# Autodesk Inventor assembly: DribblerUnit
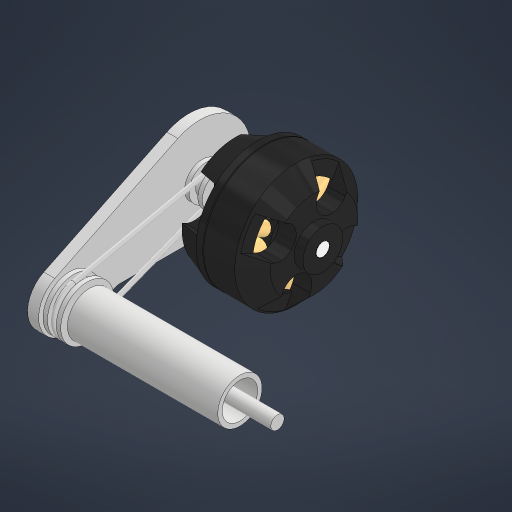
[picture p0: Inventor's stored thumbnail of the model, 512x512]
Saved by Autodesk Inventor 2024.2 (Build 282272000, 272)
## iProperties
Created: 2023-12-27
Part Number: DribblerUnit
Document SubType Name: Assembly
Designer: Hanaoka
Author: Hanaoka
## Documents named in this file (9)
- G:\共有ドライブ\reRo\05_個人\hanaoka\inventor\DribblerUnit\DribblerUnit.iam
- G:\共有ドライブ\reRo\05_個人\hanaoka\inventor\DribblerUnit\Gear_Cover.ipt
- G:\共有ドライブ\reRo\05_個人\hanaoka\inventor\DribblerUnit\Bearing_C-FL673ZZ.ipt
- G:\共有ドライブ\reRo\05_個人\hanaoka\inventor\DribblerUnit\Shaft.ipt
- G:\共有ドライブ\reRo\05_個人\hanaoka\inventor\DribblerUnit\tube.ipt
- G:\共有ドライブ\reRo\05_個人\hanaoka\inventor\DribblerUnit\C2822 1400KV BLDC v25\C2822 1400KV BLDC v25.ipt
- G:\共有ドライブ\reRo\05_個人\hanaoka\inventor\DribblerUnit\Pulley_S.ipt
- G:\共有ドライブ\reRo\05_個人\hanaoka\inventor\DribblerUnit\Pulley_L.ipt
- G:\共有ドライブ\reRo\05_個人\hanaoka\inventor\DribblerUnit\Belt.ipt
## Components (8 placed, 8 different names)
1. Gear_Cover:1 — 挿入:1, 挿入:2, 挿入:4, 挿入:5
2. Bearing_C-FL673ZZ:1 — 挿入:1
3. Shaft:1 — 挿入:2, 挿入:3, 挿入:6
4. tube:1 — 挿入:3
5. C2822 1400KV BLDC v25:1 — 挿入:4
6. Pulley_S:1 — 挿入:5, 正接:1
7. Pulley_L:1 — 挿入:6
8. Belt:1 — 正接:1
## Relationships (7: Insert 6, Tangent 1)
- 挿入:1 [Insert]: Gear_Cover:1 ↔ Bearing_C-FL673ZZ:1
- 挿入:2 [Insert]: Gear_Cover:1 ↔ Shaft:1
- 挿入:3 [Insert] (7.5 mm): Shaft:1 ↔ tube:1
- 挿入:4 [Insert] (8 mm): Gear_Cover:1 ↔ C2822 1400KV BLDC v25:1
- 挿入:5 [Insert] (0.5 mm): Gear_Cover:1 ↔ Pulley_S:1
- 挿入:6 [Insert] (3 mm): Shaft:1 ↔ Pulley_L:1
- 正接:1 [Tangent] (0.5 mm): Pulley_S:1 ↔ Belt:1
